# Autodesk Inventor assembly: Car_Assembly
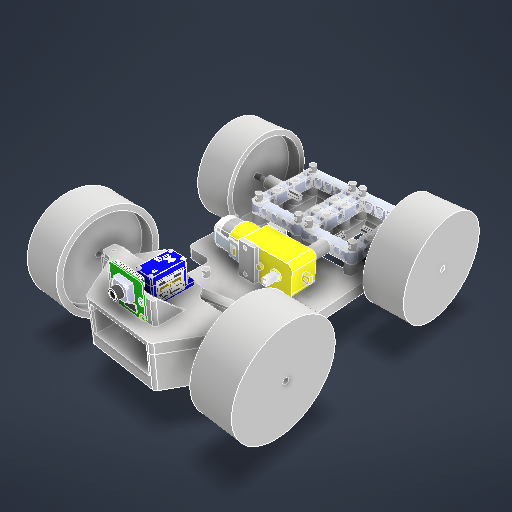
[picture p0: Inventor's stored thumbnail of the model, 512x512]
Saved by Autodesk Inventor 2025 (Build 290162000, 162)
## iProperties
Created: 2024-05-24
Part Number: Car_Assembly
Document SubType Name: Assembly
Designer: Garfieldcmix
Author: Garfieldcmix
## Documents named in this file (17)
- C:\Users\chaya\Desktop\WRO-2024-CAD\Inventor\Car_Assembly.iam
- C:\Users\chaya\Desktop\WRO-2024-CAD\Inventor\SG90 - Micro Servo 9g - Tower Pro\SG90 - Micro Servo 9g - Tower Pro.iam
- C:\Users\chaya\Desktop\WRO-2024-CAD\Inventor\Front_Bridge.ipt
- C:\Users\chaya\Desktop\WRO-2024-CAD\Inventor\SG90 - Micro Servo 9g - Tower Pro\SG90 - Micro Servo 9g - Tower Pro.2.ipt
- C:\Users\chaya\Desktop\WRO-2024-CAD\Inventor\Front_Wheel_Anchor.ipt
- C:\Users\chaya\Desktop\WRO-2024-CAD\Inventor\Front_Wheel_Anchor_MIR.ipt
- C:\Users\chaya\Desktop\WRO-2024-CAD\Inventor\Wheel.ipt
- C:\Users\chaya\Desktop\WRO-2024-CAD\Inventor\Wheel_MIR.ipt
- C:\Users\chaya\Desktop\WRO-2024-CAD\Inventor\Pi camera module3\Pi camera module3.ipt
- C:\Users\chaya\Desktop\WRO-2024-CAD\Inventor\4519 DkStone Technic Axle 3\4519 DkStone Technic Axle 3.ipt
- C:\Users\chaya\Desktop\WRO-2024-CAD\Inventor\Lego Beam Fram 5x7 (64179)\Lego Beam Fram 5x7 (64179).ipt
- C:\Users\chaya\Desktop\WRO-2024-CAD\Inventor\TT Motor\TT Motor.ipt
- C:\Users\chaya\Desktop\WRO-2024-CAD\Inventor\Lower_Chassis.ipt
- C:\Users\chaya\Desktop\WRO-2024-CAD\Inventor\Motor_Lego_Axle_Connector.ipt
- C:\Users\chaya\Desktop\WRO-2024-CAD\Inventor\Wheel_Lego_Axle_Connector.ipt
- C:\Users\chaya\Desktop\WRO-2024-CAD\Inventor\Front_Bridge_2.ipt
- C:\Users\chaya\Desktop\WRO-2024-CAD\Inventor\Servo_Steering_Linkage.ipt
## Components (23 placed, 23 different names)
1. Pi camera module3:1 — Mate:73, Mate:72, Mate:74
2. Lower_Chassis:1 — Mate:38, Mate:39, Mate:40, Mate:41, Mate:42, Mate:43, Mate:44, Mate:45, Mate:46, Mate:47, Mate:48, Mate:57, Mate:91
3. Left_Lego_Beam_Frame — Mate:37, Mate:43, Mate:44, Mate:45, Mate:50, Mate:55, Mate:60
4. Lego_Driving_Shaft_Axle — Mate:50, Mate:53, Mate:54
5. TT Motor:1 — Mate:51, Mate:52, Mate:57, Mate:91
6. Motor_Lego_Axle_Connector — Mate:51, Mate:52, Mate:53, Mate:54, Mate:55
7. Right_Lego_Beam_Frame — Mate:46, Mate:47, Mate:48, Mate:49, Mate:63
8. Left_Lego_Wheel_Axle — Mate:37, Mate:58, Mate:59
9. Left_Wheel_Lego_Axle_Connector — Mate:58, Mate:59, Mate:60, Mate:64, Flush:3
10. Left_Back_Wheel — Mate:64, Flush:3
11. Right_Lego_Wheel_Axle — Mate:49, Mate:61, Mate:62
12. Right_Wheel_Lego_Axle_Connector — Mate:61, Mate:62, Mate:63, Mate:65, Flush:4
13. Right_Back_Wheel — Mate:65, Flush:4
14. Left_Servo_Steering_Linkage — Mate:83, Mate:84, Mate:85, Mate:86
15. Right_Servo_Steering_Linkage — Mate:87, Mate:88, Mate:89, Mate:90
16. Front_Bridge:1 — Mate:38, Mate:39, Mate:40, Mate:41, Mate:42, Mate:66, Mate:67, Mate:68, Mate:75, Mate:76, Mate:79, Mate:80, Angle:1
17. Front_Bridge_2:1 — Mate:66, Mate:67, Mate:68, Mate:69, Mate:73, Mate:72, Mate:74, Mate:1, Mate:16
18. Left_Front_Wheel_Anchor — Mate:75, Mate:76, Mate:77, Mate:78, Mate:83, Mate:85, Angle:1
19. Left_Front_Wheel — Mate:77, Mate:78
20. Right_Front_Wheel_Anchor — Mate:79, Mate:80, Mate:81, Mate:82, Mate:88, Mate:89
21. Right_Front_Wheel — Mate:81, Mate:82
22. SG90_Servo [sub-assembly] — Mate:1, Mate:16, Mate:2, Mate:17, Mate:69
23. Servo_Arm — Mate:2, Mate:17, Mate:84, Mate:86, Mate:87, Mate:90
## Relationships (59: Mate 56, Flush 2, Angle 1)
- Mate:1: Front_Bridge_2:1 ↔ SG90_Servo
- Mate:16: Front_Bridge_2:1 ↔ SG90_Servo
- Mate:2: SG90_Servo ↔ Servo_Arm
- Mate:17: SG90_Servo ↔ Servo_Arm
- Mate:37: Left_Lego_Beam_Frame ↔ Left_Lego_Wheel_Axle
- Mate:38: Lower_Chassis:1 ↔ Front_Bridge:1
- Mate:39: Lower_Chassis:1 ↔ Front_Bridge:1
- Mate:40: Lower_Chassis:1 ↔ Front_Bridge:1
- Mate:41: Lower_Chassis:1 ↔ Front_Bridge:1
- Mate:42: Lower_Chassis:1 ↔ Front_Bridge:1
- Mate:43: Lower_Chassis:1 ↔ Left_Lego_Beam_Frame
- Mate:44: Lower_Chassis:1 ↔ Left_Lego_Beam_Frame
- Mate:45: Lower_Chassis:1 ↔ Left_Lego_Beam_Frame
- Mate:46: Lower_Chassis:1 ↔ Right_Lego_Beam_Frame
- Mate:47: Lower_Chassis:1 ↔ Right_Lego_Beam_Frame
- Mate:48: Lower_Chassis:1 ↔ Right_Lego_Beam_Frame
- Mate:49: Right_Lego_Beam_Frame ↔ Right_Lego_Wheel_Axle
- Mate:50: Left_Lego_Beam_Frame ↔ Lego_Driving_Shaft_Axle
- Mate:51: TT Motor:1 ↔ Motor_Lego_Axle_Connector
- Mate:52: TT Motor:1 ↔ Motor_Lego_Axle_Connector
- Mate:53: Lego_Driving_Shaft_Axle ↔ Motor_Lego_Axle_Connector
- Mate:54: Lego_Driving_Shaft_Axle ↔ Motor_Lego_Axle_Connector
- Mate:55: Left_Lego_Beam_Frame ↔ Motor_Lego_Axle_Connector
- Mate:57: Lower_Chassis:1 ↔ TT Motor:1
- Mate:58: Left_Lego_Wheel_Axle ↔ Left_Wheel_Lego_Axle_Connector
- Mate:59: Left_Lego_Wheel_Axle ↔ Left_Wheel_Lego_Axle_Connector
- Mate:60: Left_Lego_Beam_Frame ↔ Left_Wheel_Lego_Axle_Connector
- Mate:61: Right_Lego_Wheel_Axle ↔ Right_Wheel_Lego_Axle_Connector
- Mate:62: Right_Lego_Wheel_Axle ↔ Right_Wheel_Lego_Axle_Connector
- Mate:63: Right_Lego_Beam_Frame ↔ Right_Wheel_Lego_Axle_Connector
- Mate:64: Left_Wheel_Lego_Axle_Connector ↔ Left_Back_Wheel
- Flush:3: Left_Wheel_Lego_Axle_Connector ↔ Left_Back_Wheel
- Mate:65: Right_Wheel_Lego_Axle_Connector ↔ Right_Back_Wheel
- Flush:4: Right_Wheel_Lego_Axle_Connector ↔ Right_Back_Wheel
- Mate:66: Front_Bridge:1 ↔ Front_Bridge_2:1
- Mate:67: Front_Bridge:1 ↔ Front_Bridge_2:1
- Mate:68: Front_Bridge:1 ↔ Front_Bridge_2:1
- Mate:69: Front_Bridge_2:1 ↔ SG90_Servo
- Mate:73: Pi camera module3:1 ↔ Front_Bridge_2:1
- Mate:72: Pi camera module3:1 ↔ Front_Bridge_2:1
- Mate:74: Pi camera module3:1 ↔ Front_Bridge_2:1
- Mate:75: Front_Bridge:1 ↔ Left_Front_Wheel_Anchor
- Mate:76: Front_Bridge:1 ↔ Left_Front_Wheel_Anchor
- Mate:77: Left_Front_Wheel_Anchor ↔ Left_Front_Wheel
- Mate:78: Left_Front_Wheel_Anchor ↔ Left_Front_Wheel
- Mate:79: Front_Bridge:1 ↔ Right_Front_Wheel_Anchor
- Mate:80: Front_Bridge:1 ↔ Right_Front_Wheel_Anchor
- Mate:81: Right_Front_Wheel_Anchor ↔ Right_Front_Wheel
- Mate:82: Right_Front_Wheel_Anchor ↔ Right_Front_Wheel
- Mate:83: Left_Servo_Steering_Linkage ↔ Left_Front_Wheel_Anchor
- Mate:84: Left_Servo_Steering_Linkage ↔ Servo_Arm
- Mate:85: Left_Servo_Steering_Linkage ↔ Left_Front_Wheel_Anchor
- Angle:1 (180 deg): Front_Bridge:1 ↔ Left_Front_Wheel_Anchor
- Mate:86: Left_Servo_Steering_Linkage ↔ Servo_Arm
- Mate:87: Right_Servo_Steering_Linkage ↔ Servo_Arm
- Mate:88: Right_Servo_Steering_Linkage ↔ Right_Front_Wheel_Anchor
- Mate:89: Right_Servo_Steering_Linkage ↔ Right_Front_Wheel_Anchor
- Mate:90: Right_Servo_Steering_Linkage ↔ Servo_Arm
- Mate:91: Lower_Chassis:1 ↔ TT Motor:1
